# Autodesk Inventor assembly: Assembly
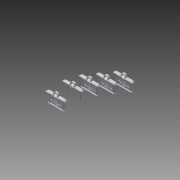
[picture p0: Inventor's stored thumbnail of the model, 180x180]
Saved by Autodesk Inventor 2018 (Build 220112000, 112)
## iProperties
Created: 2017-12-08
Part Number: Assembly
Document SubType Name: Assembly
Designer: Rus
Author: Rus
## Documents named in this file (8)
- E:\Libraries\Documents\3D Models\2017 TN Tech Ornament\Split No LED\Assembly.iam
- E:\Libraries\Documents\3D Models\2017 TN Tech Ornament\Split No LED\3D Printed2.ipt
- E:\Libraries\Documents\3D Models\2017 TN Tech Ornament\Split No LED\3D Printed2 Text.ipt
- E:\Libraries\Documents\3D Models\2017 TN Tech Ornament\Split No LED\3D Printed2 Top.ipt
- E:\Libraries\Documents\3D Models\2017 TN Tech Ornament\Split No LED\3D Printed2 Base.ipt
- E:\Libraries\Documents\3D Models\2017 TN Tech Ornament\Split No LED\3D Printed2 Eagle.ipt
- E:\Libraries\Documents\3D Models\2017 TN Tech Ornament\Split No LED\3D Printed2 Mid.ipt
- E:\Libraries\Documents\3D Models\2017 TN Tech Ornament\Split No LED\3D Printed2 Pillar R.ipt
## Components (7 placed, 7 different names)
1. 3D Printed2:1
2. 3D Printed2 Text:1 — Flush:1, Mate:1, Mate:3, Angle:2
3. 3D Printed2 Top:1 — Flush:1, Mate:1, Mate:2, Angle:1, Mate:4, Mate:5, Flush:3
4. 3D Printed2 Base:1
5. 3D Printed2 Eagle:1
6. 3D Printed2 Mid:1
7. 3D Printed2 Pillar R:1 — Mate:4, Mate:5, Flush:3
## Relationships (10: Mate 5, Flush 3, Angle 2)
- Flush:1: 3D Printed2 Text:1 ↔ 3D Printed2 Top:1
- Mate:1: 3D Printed2 Text:1 ↔ 3D Printed2 Top:1
- Mate:2: 3D Printed2 Top:1
- Angle:1 (0 deg): 3D Printed2 Top:1
- Mate:3: 3D Printed2 Text:1
- Angle:2 (0 deg): 3D Printed2 Text:1
- Flush:2
- Mate:4: 3D Printed2 Top:1 ↔ 3D Printed2 Pillar R:1
- Mate:5: 3D Printed2 Top:1 ↔ 3D Printed2 Pillar R:1
- Flush:3: 3D Printed2 Top:1 ↔ 3D Printed2 Pillar R:1
